# Autodesk Inventor assembly: FrontBumper_Assembly_MIR
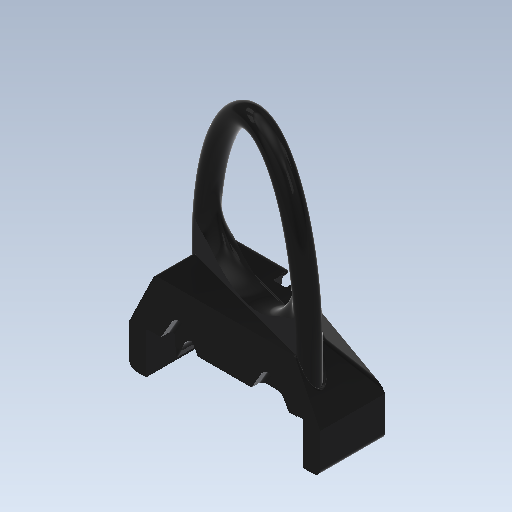
[picture p0: Inventor's stored thumbnail of the model, 512x512]
Saved by Autodesk Inventor 2020 (Build 240168000, 168)
## iProperties
Created: 2019-05-01
Part Number: FrontBumper_Assembly_MIR
Material: 一般
Document SubType Name: Assembly
Designer: taka
Author: taka
## Documents named in this file (3)
- C:\Users\6343y\Documents\Inventor\GankenKun\OpenPlatform_ver3_0\上半身\胴体\FrontBumper_MIR.iam
- C:\Users\6343y\Documents\Inventor\GankenKun\OpenPlatform_ver3_0\上半身\胴体\FreundBumper_Stand_MIR.ipt
- C:\Users\6343y\Documents\Inventor\GankenKun\OpenPlatform_ver3_0\上半身\胴体\FrontBumper_main.ipt
## Components (2 placed, 2 different names)
1. FreundBumper_Stand_MIR:1 — メイト:1, 角度:1, フラッシュ:1
2. FrontBumper_main:1 — メイト:1, 角度:1, フラッシュ:1
## Relationships (3: Mate 1, Angle 1, Flush 1)
- メイト:1 [Mate]: FreundBumper_Stand_MIR:1 ↔ FrontBumper_main:1
- 角度:1 [Angle] (180 deg): FreundBumper_Stand_MIR:1 ↔ FrontBumper_main:1
- フラッシュ:1 [Flush]: FreundBumper_Stand_MIR:1 ↔ FrontBumper_main:1
